# Autodesk Inventor assembly: Assembly3
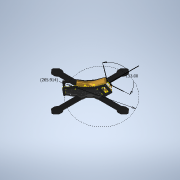
[picture p0: Inventor's stored thumbnail of the model, 180x180]
Saved by Autodesk Inventor 2020 (Build 240168000, 168)
## iProperties
Created: 2022-05-23
Part Number: Assembly3
Document SubType Name: Assembly
Designer: Steven
Author: Steven
## Documents named in this file (12)
- Y:\FPV drone stuff\0 Street League\Frames\PB-Kauri-X\3D prints\35 mm canopy\work in progress prints\session mounts\Assembly3.iam
- Y:\FPV drone stuff\0 Street League\Frames\PB-Kauri-X\Kauri arm.ipt
- Y:\FPV drone stuff\0 Street League\Frames\PB-Kauri-X\Kauri bottom plate.ipt
- Y:\FPV drone stuff\0 Street League\Frames\PB-Kauri-X\Kauri mid plate v2.ipt
- Y:\FPV drone stuff\0 Street League\Frames\PB-Kauri-X\3D prints\35 mm canopy\KauriFrontLink 35mm.ipt
- Y:\FPV drone stuff\0 Street League\Frames\PB-Kauri-X\3D prints\35 mm canopy\KauriRearLink 35mm no brass insert.ipt
- Y:\FPV drone stuff\0 Street League\Frames\PB-Kauri-X\Kauri side plate.ipt
- Y:\FPV drone stuff\0 Street League\Frames\PB-Kauri-X\3D prints\35 mm canopy\work in progress prints\Camera mounts\35mm standoff.ipt
- Y:\FPV drone stuff\0 Street League\Frames\PB-Kauri-X\3D prints\35 mm canopy\KauriCanopy Pb.ipt
- Y:\FPV drone stuff\0 Street League\Frames\PB-Kauri-X\3D prints\35 mm canopy\Kauri modular camera mount HDzero micro v1.ipt
- Y:\FPV drone stuff\0 Street League\Frames\PB-Kauri-X\3D prints\35 mm canopy\work in progress prints\Camera mounts\HDzero micro dummy.ipt
- Y:\FPV drone stuff\0 Street League\Frames\PB-Kauri-X\3D prints\35 mm canopy\Kauri modular camera mount spacer micro outside.ipt
## Components (18 placed, 11 different names)
1. Kauri arm:1 — Flush:1, Mate:4, Mate:5, Mate:12
2. Kauri arm:2 — Flush:2, Mate:6, Mate:7
3. Kauri arm:3 — Flush:3, Mate:8, Mate:9
4. Kauri arm:4 — Flush:1, Flush:2, Flush:3, Mate:1, Mate:2, Mate:3, Mate:10, Mate:11
5. Kauri bottom plate:1 — Mate:1, Mate:2, Mate:3, Mate:4, Mate:5, Mate:6, Mate:7, Mate:8, Mate:9
6. Kauri mid plate v2:1 — Mate:10, Mate:11, Mate:12, Mate:13, Mate:14, Mate:15, Mate:16, Mate:17, Mate:18
7. KauriFrontLink 35mm:1 — Mate:13, Mate:14, Mate:15, Mate:19, Mate:20, Mate:22
8. KauriRearLink 35mm no brass insert:1 — Mate:16, Mate:17, Mate:18, Mate:24
9. Kauri side plate:1 — Mate:19, Mate:20, Mate:21, Mate:23, Mate:25, Mate:27, Mate:43
10. Kauri side plate:2 — Mate:21, Mate:22, Mate:23, Mate:24, Mate:26, Mate:28, Mate:29, Mate:30, Mate:31
11. 35mm standoff:1 — Mate:25, Mate:26, Mate:41, Mate:48
12. 35mm standoff:2 — Mate:27, Mate:28, Mate:40, Mate:42, Mate:49
13. KauriCanopy Pb:1 — Mate:29, Mate:30, Mate:31
14. Kauri modular camera mount HDzero micro v1:1 — Mate:33, Mate:34, Mate:42, Mate:43, Mate:51
15. Kauri modular camera mount HDzero micro v1:2 — Mate:38, Mate:39, Mate:40, Mate:41, Mate:50
16. HDzero micro dummy:1 — Mate:33, Mate:34, Mate:38, Mate:39
17. Kauri modular camera mount spacer micro outside:1 — Mate:46, Mate:47, Mate:51
18. Kauri modular camera mount spacer micro outside:2 — Mate:46, Mate:47, Mate:48, Mate:49, Mate:50
## Relationships (48: Mate 45, Flush 3)
- Flush:1: Kauri arm:1 ↔ Kauri arm:4
- Flush:2: Kauri arm:2 ↔ Kauri arm:4
- Flush:3: Kauri arm:3 ↔ Kauri arm:4
- Mate:1: Kauri arm:4 ↔ Kauri bottom plate:1
- Mate:2: Kauri arm:4 ↔ Kauri bottom plate:1
- Mate:3: Kauri arm:4 ↔ Kauri bottom plate:1
- Mate:4: Kauri arm:1 ↔ Kauri bottom plate:1
- Mate:5: Kauri arm:1 ↔ Kauri bottom plate:1
- Mate:6: Kauri arm:2 ↔ Kauri bottom plate:1
- Mate:7: Kauri arm:2 ↔ Kauri bottom plate:1
- Mate:8: Kauri arm:3 ↔ Kauri bottom plate:1
- Mate:9: Kauri arm:3 ↔ Kauri bottom plate:1
- Mate:10: Kauri arm:4 ↔ Kauri mid plate v2:1
- Mate:11: Kauri arm:4 ↔ Kauri mid plate v2:1
- Mate:12: Kauri arm:1 ↔ Kauri mid plate v2:1
- Mate:13: Kauri mid plate v2:1 ↔ KauriFrontLink 35mm:1
- Mate:14: Kauri mid plate v2:1 ↔ KauriFrontLink 35mm:1
- Mate:15: Kauri mid plate v2:1 ↔ KauriFrontLink 35mm:1
- Mate:16: Kauri mid plate v2:1 ↔ KauriRearLink 35mm no brass insert:1
- Mate:17: Kauri mid plate v2:1 ↔ KauriRearLink 35mm no brass insert:1
- Mate:18: Kauri mid plate v2:1 ↔ KauriRearLink 35mm no brass insert:1
- Mate:19: KauriFrontLink 35mm:1 ↔ Kauri side plate:1
- Mate:20: KauriFrontLink 35mm:1 ↔ Kauri side plate:1
- Mate:21 (35 mm): Kauri side plate:1 ↔ Kauri side plate:2
- Mate:22: KauriFrontLink 35mm:1 ↔ Kauri side plate:2
- Mate:23: Kauri side plate:1 ↔ Kauri side plate:2
- Mate:24: KauriRearLink 35mm no brass insert:1 ↔ Kauri side plate:2
- Mate:25: Kauri side plate:1 ↔ 35mm standoff:1
- Mate:26: Kauri side plate:2 ↔ 35mm standoff:1
- Mate:27: Kauri side plate:1 ↔ 35mm standoff:2
- Mate:28: Kauri side plate:2 ↔ 35mm standoff:2
- Mate:29: Kauri side plate:2 ↔ KauriCanopy Pb:1
- Mate:30: Kauri side plate:2 ↔ KauriCanopy Pb:1
- Mate:31: Kauri side plate:2 ↔ KauriCanopy Pb:1
- Mate:33: Kauri modular camera mount HDzero micro v1:1 ↔ HDzero micro dummy:1
- Mate:34: Kauri modular camera mount HDzero micro v1:1 ↔ HDzero micro dummy:1
- Mate:38: Kauri modular camera mount HDzero micro v1:2 ↔ HDzero micro dummy:1
- Mate:39: Kauri modular camera mount HDzero micro v1:2 ↔ HDzero micro dummy:1
- Mate:40: 35mm standoff:2 ↔ Kauri modular camera mount HDzero micro v1:2
- Mate:41: 35mm standoff:1 ↔ Kauri modular camera mount HDzero micro v1:2
- Mate:42: 35mm standoff:2 ↔ Kauri modular camera mount HDzero micro v1:1
- Mate:43 (3.95 mm): Kauri side plate:1 ↔ Kauri modular camera mount HDzero micro v1:1
- Mate:46: Kauri modular camera mount spacer micro outside:1 ↔ Kauri modular camera mount spacer micro outside:2
- Mate:47: Kauri modular camera mount spacer micro outside:1 ↔ Kauri modular camera mount spacer micro outside:2
- Mate:48: 35mm standoff:1 ↔ Kauri modular camera mount spacer micro outside:2
- Mate:49: 35mm standoff:2 ↔ Kauri modular camera mount spacer micro outside:2
- Mate:50: Kauri modular camera mount HDzero micro v1:2 ↔ Kauri modular camera mount spacer micro outside:2
- Mate:51: Kauri modular camera mount HDzero micro v1:1 ↔ Kauri modular camera mount spacer micro outside:1
